# Autodesk Inventor assembly: Robot Assembly - 6 wheel - toughbox mini - 26x28 screwed up by climber
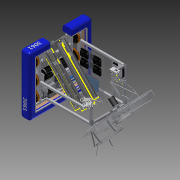
[picture p0: Inventor's stored thumbnail of the model, 180x180]
Saved by Autodesk Inventor 2013 (Build 170138000, 138)
## iProperties
Created: 2013-01-06
Part Number: Robot Assembly - 6 wheel - toughbox mini - 26x28 screwed up by climber
Document SubType Name: Assembly
Designer: Moses
Mass: 43228.5 g
Surface Area: 119845 cm^2
Volume: 41346.3 cm^3
Density: 1.04552 g/cm^3
Author: Moses
## Documents named in this file (40)
- C:\Users\Moses\Documents\GitHub\frc2013CAD\Robot Assembly - 6 wheel - toughbox mini - 26x28 screwed up by climber.iam
- C:\Users\Moses\Documents\GitHub\frc2013CAD\Drivetrain\Bearings\fr8zz-hex.ipt
- C:\Users\Moses\Documents\GitHub\frc2013CAD\Drivetrain\Drive Wheel Assembly V2.iam
- C:\Users\Moses\Documents\GitHub\frc2013CAD\Drivetrain\Standard Wheel Assembly V2.iam
- C:\Users\Moses\Documents\GitHub\frc2013CAD\Drivetrain\Toughbox-mini\Toughbox-mini-hex-long.iam
- C:\Users\Moses\Documents\GitHub\frc2013CAD\Drivetrain\6157K140 Shaft Collar\6157K140.ipt
- C:\Users\Moses\Documents\GitHub\frc2013CAD\Drivetrain\Shaft Spacer Part1.ipt
- C:\Users\Moses\Documents\GitHub\frc2013CAD\Drivetrain\Shaft Spacer Part2.ipt
- C:\Users\Moses\Documents\GitHub\frc2013CAD\Drivetrain\Shaft Spacer Part3.ipt
- C:\Users\Moses\Documents\GitHub\frc2013CAD\Drivetrain\Shaft Spacer Part4.ipt
- C:\Users\Moses\Documents\GitHub\frc2013CAD\Drivetrain\Shaft Spacer Part5.ipt
- C:\Users\Moses\Documents\GitHub\frc2013CAD\Drivetrain\Shaft Spacer Part6.ipt
- C:\Users\Moses\Documents\GitHub\frc2013CAD\Electrical\ELEC_Battery_NP18-12B.iam
- C:\Users\Moses\Documents\GitHub\frc2013CAD\Drivetrain\6061K130 Shaft\6061K130.ipt
- C:\Users\Moses\Documents\GitHub\frc2013CAD\Electrical\ELEC_CircuitBreaker_CB185-120.iam
- C:\Users\Moses\Documents\GitHub\frc2013CAD\Electrical\CS_PowerBoard_A003206.ipt
- C:\Users\Moses\Documents\GitHub\frc2013CAD\Electrical\CS_compactRIO_cRIO-FRC-II.ipt
- C:\Users\Moses\Documents\GitHub\frc2013CAD\Electrical\CS_WirelessBridge_DAP1522.ipt
- C:\Users\Moses\Documents\GitHub\frc2013CAD\Electrical\CS_Converter_CLL25-24S05.ipt
- C:\Users\Moses\Documents\GitHub\frc2013CAD\Electrical\Talon.ipt
- C:\Users\Moses\Documents\GitHub\frc2013CAD\Drivetrain\Pneumatic_Compressor_VIAIR_00090\Pneumatic_Compressor_VIAIR_00090.iam
- C:\Users\Moses\Documents\GitHub\frc2013CAD\Drivetrain\Mounting Bracket V1.500 - (toughbox-mini - sheet metal).ipt
- C:\Users\Moses\Documents\GitHub\frc2013CAD\Drivetrain\Mounting Bracket V1.500 - (toughbox-mini - sheet metal - underside).ipt
- C:\Users\Moses\Documents\GitHub\frc2013CAD\Drivetrain\Bearing Block V1.500 Drivetrain.ipt
- C:\Users\Moses\Documents\GitHub\frc2013CAD\Drivetrain\Shaft Mount V1.500 Drivetrain.ipt
- C:\Users\Moses\Documents\GitHub\frc2013CAD\Launcher\Shooter\Shooter Assembly v2.iam
- C:\Users\Moses\Documents\GitHub\frc2013CAD\Chassis\Chassis Assembly 26x28 Version\Chassis Assembly 26x28 Version.iam
- C:\Users\Moses\Documents\GitHub\frc2013CAD\Chassis\Bumpers\Bumpers (26x28)\Bumper Assembly1 (26x28 robot).iam
- C:\Users\Moses\Documents\GitHub\frc2013CAD\Climber rough space budget version\arm assembly mount plate.ipt
- C:\Users\Moses\Documents\GitHub\frc2013CAD\Cimber actual\main climber.iam
- C:\Users\Moses\Documents\GitHub\frc2013CAD\Electrical\Mounting Board 1.ipt
- C:\Users\Moses\Documents\GitHub\frc2013CAD\Electrical\CS_SideCar_A003333.ipt
- C:\Users\Moses\Documents\GitHub\frc2013CAD\Electrical\Mounting Board 2.ipt
- C:\Users\Moses\Documents\GitHub\frc2013CAD\Electrical\Mounting Board 3.ipt
- C:\Users\Moses\Documents\GitHub\frc2013CAD\Drivetrain\Wheel Mount Support Plate - drive wheel.ipt
- C:\Users\Moses\Documents\GitHub\frc2013CAD\Drivetrain\Wheel Mount Support Plate.ipt
- C:\Users\Moses\Documents\GitHub\frc2013CAD\Electrical\CS_Controller_216-3367.iam
- C:\Users\Moses\Documents\GitHub\frc2013CAD\Chassis\Bumpers\Bumpers (26x28)\Bumper Assembly2 (26x28 robot).iam
- C:\Users\Moses\Documents\GitHub\frc2013CAD\Chassis\Bumpers\Bumpers (26x28)\Bumper Assembly3 (26x28 robot).iam
- C:\Users\Moses\Documents\GitHub\frc2013CAD\Chassis\Bumpers\Bumpers (26x28)\Bumper Assembly4 (26x28 robot).iam
## Components (85 placed, 39 different names)
1. Chassis Assembly 26x28 Version:1 [sub-assembly] — Mate:1, Flush:1, Mate:2, Flush:4, Mate:3, Mate:4, Mate:5, Mate:8, Mate:9, Mate:10, Mate:17, Mate:18, Mate:19, Mate:20, Mate:21, Mate:26, Mate:27, Mate:28, Mate:29, Mate:34, Mate:35, Mate:36, Mate:37, Mate:42, Mate:43, Mate:44, Mate:47, Mate:48, Mate:51, Mate:52, Mate:55, Mate:83, Mate:84, Mate:85, Mate:89, Mate:98, Mate:99, Mate:100, Mate:101, Mate:115, Mate:116, Mate:117, Mate:118, Mate:119, Mate:120, Mate:125, Mate:126, Mate:127, Mate:128, Mate:129, Mate:130, Mate:132, Mate:136, Mate:141, Mate:153, Flush:17, Mate:154, Mate:155, Flush:18, Flush:156, Mate:157, Flush:158, Angle:1, Mate:159, Mate:183, Flush:161, Mate:190, Flush:162, Flush:191, Mate:193, Mate:194, Mate:195, Mate:196, Mate:197, Mate:198, Mate:199, Mate:200, Mate:201, Mate:202, Mate:203, Mate:204, Mate:205, Mate:206, Mate:207, Mate:208, Mate:209, Mate:210, Mate:211, Mate:212, Mate:213, Mate:214, Mate:215, Mate:216, Mate:217, Mate:218, Mate:219, Mate:220, Mate:221, Mate:222, Mate:223
2. arm assembly mount plate:2 — Mate:155, Flush:18, Flush:156, Mate:156, Flush:157, Flush:159
3. main climber:1 [sub-assembly] — Mate:156, Mate:158, Flush:159
4. arm assembly mount plate:3 — Mate:157, Flush:157, Flush:158, Mate:158
5. Mounting Board 1:1 — Mate:143, Mate:167, Mate:168, Mate:147, Mate:151, Mate:146, Mate:148, Mate:149, Mate:150, Mate:169, Mate:170, Mate:171, Mate:172, Mate:173, Mate:174, Mate:175, Mate:176, Mate:177, Mate:178, Mate:179, Mate:180, Mate:145, Mate:182, Flush:163, Mate:225, Mate:226, Mate:227, Mate:228, Mate:229, Mate:230, Mate:231, Mate:232, Mate:233, Mate:234, Mate:235, Mate:236, Mate:237, Mate:238, Mate:239
6. CS_SideCar_A003333:1 — Mate:184, Mate:185, Mate:186
7. Mounting Board 2:1 — Mate:183, Flush:161, Mate:184, Mate:185, Mate:186, Mate:187, Mate:142
8. Mounting Board 3:1 — Mate:190, Flush:162, Mate:16, Mate:188, Mate:189, Flush:191, Mate:144, Mate:240, Mate:241
9. Wheel Mount Support Plate - drive wheel:1 — Mate:194, Mate:195, Mate:196
10. Wheel Mount Support Plate - drive wheel:2 — Mate:197, Mate:198, Mate:199
11. Wheel Mount Support Plate:1 — Mate:200, Mate:201, Mate:202
12. Wheel Mount Support Plate:2 — Mate:203, Mate:204, Mate:205
13. Wheel Mount Support Plate:3 — Mate:206, Mate:207, Mate:208
14. Wheel Mount Support Plate:4 — Mate:209, Mate:210, Mate:211
15. Wheel Mount Support Plate:5 — Mate:212, Mate:213, Mate:214
16. Wheel Mount Support Plate:6 — Mate:215, Mate:216, Mate:217
17. Wheel Mount Support Plate:7 — Mate:218, Mate:219, Mate:220
18. Wheel Mount Support Plate:8 — Mate:221, Mate:222, Mate:223
19. CS_Controller_216-3367:3 [sub-assembly] — Mate:229, Mate:230, Mate:231
20. CS_Controller_216-3367:4 [sub-assembly] — Mate:226, Mate:227, Mate:228
21. CS_Controller_216-3367:5 [sub-assembly] — Mate:233, Mate:236, Mate:237
22. CS_Controller_216-3367:6 [sub-assembly] — Mate:232, Mate:234, Mate:235
23. Bumper Assembly1 (26x28 robot):1 [sub-assembly] — Mate:5, Mate:3, Flush:6, Flush:9, Flush:10
24. Bumper Assembly1 (26x28 robot):2 [sub-assembly] — Mate:1, Flush:1, Flush:3, Flush:2, Flush:7, Flush:8
25. Bumper Assembly2 (26x28 robot):1 [sub-assembly] — Mate:2, Flush:2, Flush:3, Flush:4, Mate:5, Flush:10
26. Bumper Assembly3 (26x28 robot):1 [sub-assembly] — Flush:9, Mate:5, Flush:6
27. Bumper Assembly4 (26x28 robot):1 [sub-assembly] — Mate:4, Flush:7, Flush:8
28. Pneumatic_Compressor_VIAIR_00090:1 [sub-assembly] — Mate:144, Mate:240, Mate:241
29. Shaft Spacer Part1:1 — Insert:111
30. Shaft Spacer Part2:1 — Insert:112
31. Shaft Spacer Part1:3 — Insert:113
32. Shaft Spacer Part2:2 — Insert:114
33. Shaft Spacer Part3:1 — Insert:115
34. Shaft Spacer Part3:2 — Insert:116
35. Shaft Spacer Part4:2 — Insert:117
36. Shaft Spacer Part4:1 — Insert:118
37. Shaft Spacer Part5:1 — Insert:119
38. Shaft Spacer Part5:2 — Insert:120
39. Shaft Spacer Part6:1 — Insert:121
40. Shaft Spacer Part6:2 — Insert:122
41. 6157K140:1 — Insert:107, Insert:113
42. 6157K140:2 — Insert:108, Insert:114
43. 6157K140:3 — Insert:110, Insert:111
44. 6157K140:4 — Insert:109, Insert:112
45. Toughbox-mini-hex-long:2 [sub-assembly] — Mate:131, Mate:132, Mate:133, Mate:134, Mate:135, Insert:118, Tangent:1
46. Toughbox-mini-hex-long:1 [sub-assembly] — Mate:136, Mate:137, Mate:138, Mate:139, Mate:140, Insert:117
47. fr8zz-hex:1 — Insert:94, Insert:116
48. Bearing Block V1.500 Drivetrain:1 — Mate:83, Mate:84, Mate:85, Insert:106
49. Bearing Block V1.500 Drivetrain:2 — Mate:98, Mate:99, Mate:100, Insert:94
50. fr8zz-hex:2 — Insert:106, Insert:115
51. Mounting Bracket V1.500 - (toughbox-mini - sheet metal):1 — Mate:115, Mate:116, Mate:117, Mate:137, Mate:138
52. Mounting Bracket V1.500 - (toughbox-mini - sheet metal):2 — Mate:118, Mate:119, Mate:120, Mate:131, Mate:133
53. Mounting Bracket V1.500 - (toughbox-mini - sheet metal - underside):1 — Mate:125, Mate:126, Mate:127
54. Mounting Bracket V1.500 - (toughbox-mini - sheet metal - underside):2 — Mate:128, Mate:129, Mate:130
55. Shaft Mount V1.500 Drivetrain:8 — Mate:34, Mate:35, Mate:51, Insert:121
56. Shaft Mount V1.500 Drivetrain:7 — Mate:28, Mate:29, Mate:48, Insert:110
57. Shaft Mount V1.500 Drivetrain:6 — Mate:42, Mate:43, Mate:47, Insert:122
58. Shaft Mount V1.500 Drivetrain:5 — Mate:36, Mate:37, Mate:44, Insert:107
59. Shaft Mount V1.500 Drivetrain:4 — Mate:26, Mate:27, Mate:55, Insert:7, Insert:109
60. Shaft Mount V1.500 Drivetrain:3 — Mate:20, Mate:21, Mate:52, Insert:5, Insert:119
61. Shaft Mount V1.500 Drivetrain:2 — Mate:17, Mate:18, Mate:19, Insert:2, Insert:108
62. Shaft Mount V1.500 Drivetrain:1 — Mate:8, Mate:9, Mate:10, Insert:1, Insert:120
63. 6061K130:4 — Insert:7, Mate:21
64. 6061K130:3 — Insert:5, Mate:22
65. 6061K130:2 — Insert:2, Mate:19, Mate:192
66. 6061K130:1 — Insert:1, Mate:17
67. Standard Wheel Assembly V2:3 [sub-assembly] — Mate:17, Flush:13, Rotation:1
68. Drive Wheel Assembly V2:1 [sub-assembly] — Mate:89, Flush:13, Flush:15, Mate:139, Mate:140, Rotation:1, Rotation:2
69. Standard Wheel Assembly V2:1 [sub-assembly] — Mate:19, Flush:15, Rotation:2
70. Standard Wheel Assembly V2:2 [sub-assembly] — Mate:21, Flush:11, Rotation:4
71. Standard Wheel Assembly V2:4 [sub-assembly] — Mate:22, Flush:12, Rotation:3
72. Drive Wheel Assembly V2:2 [sub-assembly] — Mate:101, Flush:11, Flush:12, Mate:134, Mate:135, Rotation:3, Rotation:4
73. Talon:1 — Mate:147, Mate:169, Mate:170
74. Talon:2 — Mate:151, Mate:171, Mate:172
75. Talon:3 — Mate:146, Mate:175, Mate:176
76. Talon:4 — Mate:148, Mate:173, Mate:174
77. Talon:5 — Mate:149, Mate:177, Mate:178
78. Talon:6 — Mate:150, Mate:179, Mate:180
79. CS_Converter_CLL25-24S05:1 — Mate:145, Mate:238, Mate:239
80. CS_WirelessBridge_DAP1522:1 — Flush:152, Mate:164, Mate:224
81. CS_compactRIO_cRIO-FRC-II:1 — Mate:16, Mate:188, Mate:189
82. ELEC_CircuitBreaker_CB185-120:1 [sub-assembly] — Mate:142
83. ELEC_Battery_NP18-12B:1 [sub-assembly] — Mate:141, Mate:192, Mate:193
84. CS_PowerBoard_A003206:1 — Mate:143, Mate:167, Mate:168
85. Shooter Assembly v2:1 [sub-assembly] — Mate:153, Flush:17, Mate:154, Mate:159, Mate:164, Flush:152, Mate:182, Mate:187, Mate:224, Flush:163, Mate:225
## Relationships (209: Mate 157, Flush 24, Insert 22, RelateRotation 4, Angle 1, Tangent 1)
- Mate:1: Chassis Assembly 26x28 Version:1 ↔ Bumper Assembly1 (26x28 robot):2
- Flush:1: Chassis Assembly 26x28 Version:1 ↔ Bumper Assembly1 (26x28 robot):2
- Mate:2: Chassis Assembly 26x28 Version:1 ↔ Bumper Assembly2 (26x28 robot):1
- Flush:2: Bumper Assembly1 (26x28 robot):2 ↔ Bumper Assembly2 (26x28 robot):1
- Flush:3: Bumper Assembly1 (26x28 robot):2 ↔ Bumper Assembly2 (26x28 robot):1
- Flush:4 (-69.85 mm): Chassis Assembly 26x28 Version:1 ↔ Bumper Assembly2 (26x28 robot):1
- Mate:5: Bumper Assembly1 (26x28 robot):1 ↔ Bumper Assembly2 (26x28 robot):1
- Mate:3: Chassis Assembly 26x28 Version:1 ↔ Bumper Assembly1 (26x28 robot):1
- Flush:6: Bumper Assembly1 (26x28 robot):1 ↔ Bumper Assembly3 (26x28 robot):1
- Mate:4: Chassis Assembly 26x28 Version:1 ↔ Bumper Assembly4 (26x28 robot):1
- Flush:7: Bumper Assembly1 (26x28 robot):2 ↔ Bumper Assembly4 (26x28 robot):1
- Flush:8: Bumper Assembly1 (26x28 robot):2 ↔ Bumper Assembly4 (26x28 robot):1
- Flush:9: Bumper Assembly1 (26x28 robot):1 ↔ Bumper Assembly3 (26x28 robot):1
- Flush:10: Bumper Assembly1 (26x28 robot):1 ↔ Bumper Assembly2 (26x28 robot):1
- Mate:5: Chassis Assembly 26x28 Version:1 ↔ Bumper Assembly3 (26x28 robot):1
- Insert:1 (-6.35 mm): Shaft Mount V1.500 Drivetrain:1 ↔ 6061K130:1
- Insert:2 (-6.35 mm): Shaft Mount V1.500 Drivetrain:2 ↔ 6061K130:2
- Insert:5 (-6.35 mm): Shaft Mount V1.500 Drivetrain:3 ↔ 6061K130:3
- Insert:7 (-6.35 mm): Shaft Mount V1.500 Drivetrain:4 ↔ 6061K130:4
- Mate:8: Chassis Assembly 26x28 Version:1 ↔ Shaft Mount V1.500 Drivetrain:1
- Mate:9: Chassis Assembly 26x28 Version:1 ↔ Shaft Mount V1.500 Drivetrain:1
- Mate:10: Chassis Assembly 26x28 Version:1 ↔ Shaft Mount V1.500 Drivetrain:1
- Mate:17: Chassis Assembly 26x28 Version:1 ↔ Shaft Mount V1.500 Drivetrain:2
- Mate:18: Chassis Assembly 26x28 Version:1 ↔ Shaft Mount V1.500 Drivetrain:2
- Mate:19: Chassis Assembly 26x28 Version:1 ↔ Shaft Mount V1.500 Drivetrain:2
- Mate:20: Chassis Assembly 26x28 Version:1 ↔ Shaft Mount V1.500 Drivetrain:3
- Mate:21: Chassis Assembly 26x28 Version:1 ↔ Shaft Mount V1.500 Drivetrain:3
- Mate:26: Chassis Assembly 26x28 Version:1 ↔ Shaft Mount V1.500 Drivetrain:4
- Mate:27: Chassis Assembly 26x28 Version:1 ↔ Shaft Mount V1.500 Drivetrain:4
- Mate:28: Chassis Assembly 26x28 Version:1 ↔ Shaft Mount V1.500 Drivetrain:7
- Mate:29: Chassis Assembly 26x28 Version:1 ↔ Shaft Mount V1.500 Drivetrain:7
- Mate:34: Chassis Assembly 26x28 Version:1 ↔ Shaft Mount V1.500 Drivetrain:8
- Mate:35: Chassis Assembly 26x28 Version:1 ↔ Shaft Mount V1.500 Drivetrain:8
- Mate:36: Chassis Assembly 26x28 Version:1 ↔ Shaft Mount V1.500 Drivetrain:5
- Mate:37: Chassis Assembly 26x28 Version:1 ↔ Shaft Mount V1.500 Drivetrain:5
- Mate:42: Chassis Assembly 26x28 Version:1 ↔ Shaft Mount V1.500 Drivetrain:6
- Mate:43: Chassis Assembly 26x28 Version:1 ↔ Shaft Mount V1.500 Drivetrain:6
- Mate:44: Chassis Assembly 26x28 Version:1 ↔ Shaft Mount V1.500 Drivetrain:5
- Mate:47: Chassis Assembly 26x28 Version:1 ↔ Shaft Mount V1.500 Drivetrain:6
- Mate:48: Chassis Assembly 26x28 Version:1 ↔ Shaft Mount V1.500 Drivetrain:7
- Mate:51: Chassis Assembly 26x28 Version:1 ↔ Shaft Mount V1.500 Drivetrain:8
- Mate:52: Chassis Assembly 26x28 Version:1 ↔ Shaft Mount V1.500 Drivetrain:3
- Mate:55: Chassis Assembly 26x28 Version:1 ↔ Shaft Mount V1.500 Drivetrain:4
- Mate:17: 6061K130:1 ↔ Standard Wheel Assembly V2:3
- Mate:19: 6061K130:2 ↔ Standard Wheel Assembly V2:1
- Mate:21: 6061K130:4 ↔ Standard Wheel Assembly V2:2
- Mate:22: 6061K130:3 ↔ Standard Wheel Assembly V2:4
- Mate:83: Chassis Assembly 26x28 Version:1 ↔ Bearing Block V1.500 Drivetrain:1
- Mate:84: Chassis Assembly 26x28 Version:1 ↔ Bearing Block V1.500 Drivetrain:1
- Mate:85: Chassis Assembly 26x28 Version:1 ↔ Bearing Block V1.500 Drivetrain:1
- Mate:89 (6.35 mm): Chassis Assembly 26x28 Version:1 ↔ Drive Wheel Assembly V2:1
- Insert:94: fr8zz-hex:1 ↔ Bearing Block V1.500 Drivetrain:2
- Mate:98: Chassis Assembly 26x28 Version:1 ↔ Bearing Block V1.500 Drivetrain:2
- Mate:99: Chassis Assembly 26x28 Version:1 ↔ Bearing Block V1.500 Drivetrain:2
- Mate:100: Chassis Assembly 26x28 Version:1 ↔ Bearing Block V1.500 Drivetrain:2
- Mate:101 (6.35 mm): Chassis Assembly 26x28 Version:1 ↔ Drive Wheel Assembly V2:2
- Insert:106: Bearing Block V1.500 Drivetrain:1 ↔ fr8zz-hex:2
- Mate:115: Chassis Assembly 26x28 Version:1 ↔ Mounting Bracket V1.500 - (toughbox-mini - sheet metal):1
- Mate:116: Chassis Assembly 26x28 Version:1 ↔ Mounting Bracket V1.500 - (toughbox-mini - sheet metal):1
- Mate:117: Chassis Assembly 26x28 Version:1 ↔ Mounting Bracket V1.500 - (toughbox-mini - sheet metal):1
- Mate:118: Chassis Assembly 26x28 Version:1 ↔ Mounting Bracket V1.500 - (toughbox-mini - sheet metal):2
- Mate:119: Chassis Assembly 26x28 Version:1 ↔ Mounting Bracket V1.500 - (toughbox-mini - sheet metal):2
- Mate:120: Chassis Assembly 26x28 Version:1 ↔ Mounting Bracket V1.500 - (toughbox-mini - sheet metal):2
- Flush:11: Standard Wheel Assembly V2:2 ↔ Drive Wheel Assembly V2:2
- Flush:12: Standard Wheel Assembly V2:4 ↔ Drive Wheel Assembly V2:2
- Flush:13: Standard Wheel Assembly V2:3 ↔ Drive Wheel Assembly V2:1
- Mate:125: Chassis Assembly 26x28 Version:1 ↔ Mounting Bracket V1.500 - (toughbox-mini - sheet metal - underside):1
- Mate:126: Chassis Assembly 26x28 Version:1 ↔ Mounting Bracket V1.500 - (toughbox-mini - sheet metal - underside):1
- Mate:127: Chassis Assembly 26x28 Version:1 ↔ Mounting Bracket V1.500 - (toughbox-mini - sheet metal - underside):1
- Mate:128: Chassis Assembly 26x28 Version:1 ↔ Mounting Bracket V1.500 - (toughbox-mini - sheet metal - underside):2
- Mate:129: Chassis Assembly 26x28 Version:1 ↔ Mounting Bracket V1.500 - (toughbox-mini - sheet metal - underside):2
- Mate:130: Chassis Assembly 26x28 Version:1 ↔ Mounting Bracket V1.500 - (toughbox-mini - sheet metal - underside):2
- Flush:15: Drive Wheel Assembly V2:1 ↔ Standard Wheel Assembly V2:1
- Mate:131: Toughbox-mini-hex-long:2 ↔ Mounting Bracket V1.500 - (toughbox-mini - sheet metal):2
- Mate:132: Chassis Assembly 26x28 Version:1 ↔ Toughbox-mini-hex-long:2
- Mate:133: Toughbox-mini-hex-long:2 ↔ Mounting Bracket V1.500 - (toughbox-mini - sheet metal):2
- Mate:134: Toughbox-mini-hex-long:2 ↔ Drive Wheel Assembly V2:2
- Mate:135: Toughbox-mini-hex-long:2 ↔ Drive Wheel Assembly V2:2
- Mate:136: Chassis Assembly 26x28 Version:1 ↔ Toughbox-mini-hex-long:1
- Mate:137: Toughbox-mini-hex-long:1 ↔ Mounting Bracket V1.500 - (toughbox-mini - sheet metal):1
- Mate:138: Toughbox-mini-hex-long:1 ↔ Mounting Bracket V1.500 - (toughbox-mini - sheet metal):1
- Mate:139: Toughbox-mini-hex-long:1 ↔ Drive Wheel Assembly V2:1
- Mate:140: Toughbox-mini-hex-long:1 ↔ Drive Wheel Assembly V2:1
- Rotation:1 [RelateRotation] (1 ul): Standard Wheel Assembly V2:3 ↔ Drive Wheel Assembly V2:1
- Rotation:2 [RelateRotation] (1 ul): Drive Wheel Assembly V2:1 ↔ Standard Wheel Assembly V2:1
- Rotation:3 [RelateRotation] (1 ul): Standard Wheel Assembly V2:4 ↔ Drive Wheel Assembly V2:2
- Rotation:4 [RelateRotation] (1 ul): Standard Wheel Assembly V2:2 ↔ Drive Wheel Assembly V2:2
- Insert:107: 6157K140:1 ↔ Shaft Mount V1.500 Drivetrain:5
- Insert:108: 6157K140:2 ↔ Shaft Mount V1.500 Drivetrain:2
- Insert:109: 6157K140:4 ↔ Shaft Mount V1.500 Drivetrain:4
- Insert:110: 6157K140:3 ↔ Shaft Mount V1.500 Drivetrain:7
- Insert:111: Shaft Spacer Part1:1 ↔ 6157K140:3
- Insert:112: Shaft Spacer Part2:1 ↔ 6157K140:4
- Insert:113: Shaft Spacer Part1:3 ↔ 6157K140:1
- Insert:114: Shaft Spacer Part2:2 ↔ 6157K140:2
- Insert:115: Shaft Spacer Part3:1 ↔ fr8zz-hex:2
- Insert:116: Shaft Spacer Part3:2 ↔ fr8zz-hex:1
- Insert:117: Shaft Spacer Part4:2 ↔ Toughbox-mini-hex-long:1
- Insert:118: Shaft Spacer Part4:1 ↔ Toughbox-mini-hex-long:2
- Insert:119: Shaft Spacer Part5:1 ↔ Shaft Mount V1.500 Drivetrain:3
- Insert:120: Shaft Spacer Part5:2 ↔ Shaft Mount V1.500 Drivetrain:1
- Insert:121: Shaft Spacer Part6:1 ↔ Shaft Mount V1.500 Drivetrain:8
- Insert:122: Shaft Spacer Part6:2 ↔ Shaft Mount V1.500 Drivetrain:6
- Mate:141: Chassis Assembly 26x28 Version:1 ↔ ELEC_Battery_NP18-12B:1
- Mate:142: Mounting Board 2:1 ↔ ELEC_CircuitBreaker_CB185-120:1
- Mate:143: Mounting Board 1:1 ↔ CS_PowerBoard_A003206:1
- Mate:16: Mounting Board 3:1 ↔ CS_compactRIO_cRIO-FRC-II:1
- Mate:144: Mounting Board 3:1 ↔ Pneumatic_Compressor_VIAIR_00090:1
- Mate:145: Mounting Board 1:1 ↔ CS_Converter_CLL25-24S05:1
- Mate:146: Mounting Board 1:1 ↔ Talon:3
- Mate:147: Mounting Board 1:1 ↔ Talon:1
- Mate:148: Mounting Board 1:1 ↔ Talon:4
- Mate:149: Mounting Board 1:1 ↔ Talon:5
- Mate:150: Mounting Board 1:1 ↔ Talon:6
- Mate:151: Mounting Board 1:1 ↔ Talon:2
- Flush:152: CS_WirelessBridge_DAP1522:1 ↔ Shooter Assembly v2:1
- Mate:153: Chassis Assembly 26x28 Version:1 ↔ Shooter Assembly v2:1
- Flush:17: Chassis Assembly 26x28 Version:1 ↔ Shooter Assembly v2:1
- Mate:154: Chassis Assembly 26x28 Version:1 ↔ Shooter Assembly v2:1
- Mate:155: Chassis Assembly 26x28 Version:1 ↔ arm assembly mount plate:2
- Flush:18: Chassis Assembly 26x28 Version:1 ↔ arm assembly mount plate:2
- Flush:156 (44.45 mm): Chassis Assembly 26x28 Version:1 ↔ arm assembly mount plate:2
- Mate:156: arm assembly mount plate:2 ↔ main climber:1
- Mate:157: Chassis Assembly 26x28 Version:1 ↔ arm assembly mount plate:3
- Flush:157: arm assembly mount plate:2 ↔ arm assembly mount plate:3
- Flush:158: Chassis Assembly 26x28 Version:1 ↔ arm assembly mount plate:3
- Mate:158: main climber:1 ↔ arm assembly mount plate:3
- Flush:159 (-22.9616 mm): arm assembly mount plate:2 ↔ main climber:1
- Angle:1 (0 deg): Chassis Assembly 26x28 Version:1
- Tangent:1: Toughbox-mini-hex-long:2
- Mate:159: Chassis Assembly 26x28 Version:1 ↔ Shooter Assembly v2:1
- Mate:164: CS_WirelessBridge_DAP1522:1 ↔ Shooter Assembly v2:1
- Mate:167: Mounting Board 1:1 ↔ CS_PowerBoard_A003206:1
- Mate:168: Mounting Board 1:1 ↔ CS_PowerBoard_A003206:1
- Mate:169: Mounting Board 1:1 ↔ Talon:1
- Mate:170: Mounting Board 1:1 ↔ Talon:1
- Mate:171: Mounting Board 1:1 ↔ Talon:2
- Mate:172: Mounting Board 1:1 ↔ Talon:2
- Mate:173: Mounting Board 1:1 ↔ Talon:4
- Mate:174: Mounting Board 1:1 ↔ Talon:4
- Mate:175: Mounting Board 1:1 ↔ Talon:3
- Mate:176: Mounting Board 1:1 ↔ Talon:3
- Mate:177: Mounting Board 1:1 ↔ Talon:5
- Mate:178: Mounting Board 1:1 ↔ Talon:5
- Mate:179: Mounting Board 1:1 ↔ Talon:6
- Mate:180: Mounting Board 1:1 ↔ Talon:6
- Mate:182 (50.8 mm): Mounting Board 1:1 ↔ Shooter Assembly v2:1
- Mate:183 (101.6 mm): Chassis Assembly 26x28 Version:1 ↔ Mounting Board 2:1
- Flush:161: Chassis Assembly 26x28 Version:1 ↔ Mounting Board 2:1
- Mate:184: CS_SideCar_A003333:1 ↔ Mounting Board 2:1
- Mate:185: CS_SideCar_A003333:1 ↔ Mounting Board 2:1
- Mate:186: CS_SideCar_A003333:1 ↔ Mounting Board 2:1
- Mate:187: Mounting Board 2:1 ↔ Shooter Assembly v2:1
- Mate:188: Mounting Board 3:1 ↔ CS_compactRIO_cRIO-FRC-II:1
- Mate:189: Mounting Board 3:1 ↔ CS_compactRIO_cRIO-FRC-II:1
- Mate:190: Chassis Assembly 26x28 Version:1 ↔ Mounting Board 3:1
- Flush:162: Chassis Assembly 26x28 Version:1 ↔ Mounting Board 3:1
- Flush:191: Chassis Assembly 26x28 Version:1 ↔ Mounting Board 3:1
- Mate:192: 6061K130:2 ↔ ELEC_Battery_NP18-12B:1
- Mate:193 (25.4 mm): Chassis Assembly 26x28 Version:1 ↔ ELEC_Battery_NP18-12B:1
- Mate:194: Chassis Assembly 26x28 Version:1 ↔ Wheel Mount Support Plate - drive wheel:1
- Mate:195: Chassis Assembly 26x28 Version:1 ↔ Wheel Mount Support Plate - drive wheel:1
- Mate:196: Chassis Assembly 26x28 Version:1 ↔ Wheel Mount Support Plate - drive wheel:1
- Mate:197: Chassis Assembly 26x28 Version:1 ↔ Wheel Mount Support Plate - drive wheel:2
- Mate:198: Chassis Assembly 26x28 Version:1 ↔ Wheel Mount Support Plate - drive wheel:2
- Mate:199: Chassis Assembly 26x28 Version:1 ↔ Wheel Mount Support Plate - drive wheel:2
- Mate:200: Chassis Assembly 26x28 Version:1 ↔ Wheel Mount Support Plate:1
- Mate:201: Chassis Assembly 26x28 Version:1 ↔ Wheel Mount Support Plate:1
- Mate:202: Chassis Assembly 26x28 Version:1 ↔ Wheel Mount Support Plate:1
- Mate:203: Chassis Assembly 26x28 Version:1 ↔ Wheel Mount Support Plate:2
- Mate:204: Chassis Assembly 26x28 Version:1 ↔ Wheel Mount Support Plate:2
- Mate:205: Chassis Assembly 26x28 Version:1 ↔ Wheel Mount Support Plate:2
- Mate:206: Chassis Assembly 26x28 Version:1 ↔ Wheel Mount Support Plate:3
- Mate:207: Chassis Assembly 26x28 Version:1 ↔ Wheel Mount Support Plate:3
- Mate:208: Chassis Assembly 26x28 Version:1 ↔ Wheel Mount Support Plate:3
- Mate:209: Chassis Assembly 26x28 Version:1 ↔ Wheel Mount Support Plate:4
- Mate:210: Chassis Assembly 26x28 Version:1 ↔ Wheel Mount Support Plate:4
- Mate:211: Chassis Assembly 26x28 Version:1 ↔ Wheel Mount Support Plate:4
- Mate:212: Chassis Assembly 26x28 Version:1 ↔ Wheel Mount Support Plate:5
- Mate:213: Chassis Assembly 26x28 Version:1 ↔ Wheel Mount Support Plate:5
- Mate:214: Chassis Assembly 26x28 Version:1 ↔ Wheel Mount Support Plate:5
- Mate:215: Chassis Assembly 26x28 Version:1 ↔ Wheel Mount Support Plate:6
- Mate:216: Chassis Assembly 26x28 Version:1 ↔ Wheel Mount Support Plate:6
- Mate:217: Chassis Assembly 26x28 Version:1 ↔ Wheel Mount Support Plate:6
- Mate:218: Chassis Assembly 26x28 Version:1 ↔ Wheel Mount Support Plate:7
- Mate:219: Chassis Assembly 26x28 Version:1 ↔ Wheel Mount Support Plate:7
- Mate:220: Chassis Assembly 26x28 Version:1 ↔ Wheel Mount Support Plate:7
- Mate:221: Chassis Assembly 26x28 Version:1 ↔ Wheel Mount Support Plate:8
- Mate:222: Chassis Assembly 26x28 Version:1 ↔ Wheel Mount Support Plate:8
- Mate:223: Chassis Assembly 26x28 Version:1 ↔ Wheel Mount Support Plate:8
- Mate:224: CS_WirelessBridge_DAP1522:1 ↔ Shooter Assembly v2:1
- Flush:163: Mounting Board 1:1 ↔ Shooter Assembly v2:1
- Mate:225 (50.8 mm): Mounting Board 1:1 ↔ Shooter Assembly v2:1
- Mate:226: Mounting Board 1:1 ↔ CS_Controller_216-3367:4
- Mate:227: Mounting Board 1:1 ↔ CS_Controller_216-3367:4
- Mate:228: Mounting Board 1:1 ↔ CS_Controller_216-3367:4
- Mate:229: Mounting Board 1:1 ↔ CS_Controller_216-3367:3
- Mate:230: Mounting Board 1:1 ↔ CS_Controller_216-3367:3
- Mate:231: Mounting Board 1:1 ↔ CS_Controller_216-3367:3
- Mate:232: Mounting Board 1:1 ↔ CS_Controller_216-3367:6
- Mate:233: Mounting Board 1:1 ↔ CS_Controller_216-3367:5
- Mate:234: Mounting Board 1:1 ↔ CS_Controller_216-3367:6
- Mate:235: Mounting Board 1:1 ↔ CS_Controller_216-3367:6
- Mate:236: Mounting Board 1:1 ↔ CS_Controller_216-3367:5
- Mate:237: Mounting Board 1:1 ↔ CS_Controller_216-3367:5
- Mate:238: Mounting Board 1:1 ↔ CS_Converter_CLL25-24S05:1
- Mate:239: Mounting Board 1:1 ↔ CS_Converter_CLL25-24S05:1
- Mate:240: Mounting Board 3:1 ↔ Pneumatic_Compressor_VIAIR_00090:1
- Mate:241: Mounting Board 3:1 ↔ Pneumatic_Compressor_VIAIR_00090:1
